# Autodesk Inventor assembly: LinearClampingHub
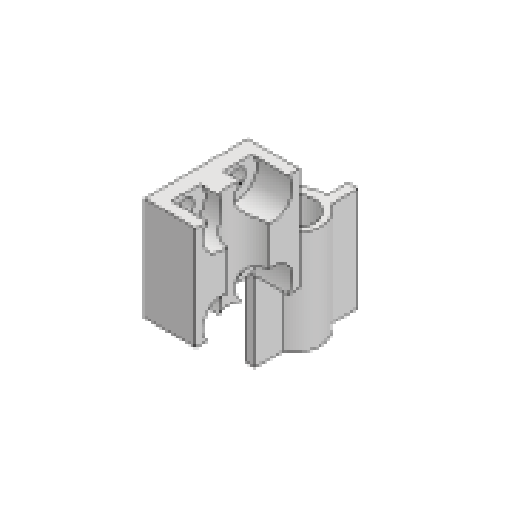
[picture p0: Inventor's stored thumbnail of the model, 512x512]
Saved by Autodesk Inventor 2023 (Build 270158000, 158)
## iProperties
Created: 2022-10-30
Part Number: LinearClampingHub
Document SubType Name: Assembly
Designer: deli
Author: deli
## Documents named in this file (3)
- C:\Users\deli\OneDrive - Eastside Preparatory School\FTC\8103-power-play\CAD\LinearClampingHub.iam
- C:\Users\deli\OneDrive - Eastside Preparatory School\FTC\8103-power-play\CAD\LinearClampPart2.ipt
- C:\Users\deli\OneDrive - Eastside Preparatory School\FTC\8103-power-play\CAD\LinearClamp.ipt
## Components (2 placed, 2 different names)
1. LinearClampPart2:1 — Mate:1, Mate:2
2. LinearClamp:1 — Mate:1, Mate:2
## Relationships (2: Mate 2)
- Mate:1: LinearClampPart2:1 ↔ LinearClamp:1
- Mate:2: LinearClampPart2:1 ↔ LinearClamp:1
